# Autodesk Inventor assembly: sweeper
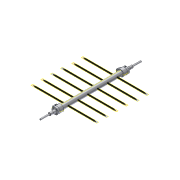
[picture p0: Inventor's stored thumbnail of the model, 180x180]
Saved by Autodesk Inventor 2015 SP1 (Build 190203100, 203)
## iProperties
Created: 2015-01-25
Part Number: sweeper
Document SubType Name: Assembly
Designer: rihoobler
Author: rihoobler
## Documents named in this file (8)
- C:\Users\datenney\Documents\GitHub\CAD\SerenityMk.2\sweeper.iam
- C:\Users\datenney\Documents\GitHub\CAD\SerenityMk.2\Sweeper tube.ipt
- C:\Users\datenney\Documents\GitHub\CAD\SerenityMk.2\Imported Components\tetrix_739077_2012\tetrix_739077_2012.ipt
- C:\Users\datenney\Documents\GitHub\CAD\SerenityMk.2\Imported Components\tetrix_739172_2012\tetrix_739172_2012.iam
- C:\Users\datenney\Documents\GitHub\CAD\SerenityMk.2\Imported Components\tetrix_739088_2012\tetrix_739088_2012.ipt
- C:\Users\datenney\Documents\GitHub\CAD\SerenityMk.2\Imported Components\tetrix_739101_2012\tetrix_739101_2012.ipt
- C:\Users\datenney\Documents\GitHub\CAD\SerenityMk.2\Imported Components\tetrix_739068_2012_288_channel\Part1.ipt
- C:\Users\datenney\Documents\GitHub\CAD\SerenityMk.2\Zip tie start.ipt
## Components (24 placed, 7 different names)
1. Sweeper tube:1 — Insert:1, Insert:2, Mate:40, Mate:47
2. tetrix_739077_2012:1 — Insert:2, Insert:4, Flush:42, Mate:45
3. tetrix_739077_2012:2 — Insert:1, Insert:3, Mate:41, Flush:42, Mate:48, Angle:7, Flush:43
4. tetrix_739172_2012:1 [sub-assembly] — Insert:4, Mate:15, Flush:3, Insert:7, Mate:45
5. tetrix_739172_2012:2 [sub-assembly] — Insert:3, Mate:16, Flush:4, Insert:5, Mate:48
6. tetrix_739088_2012:1 — Mate:16, Flush:4, Angle:7, Angle:8
7. tetrix_739088_2012:2 — Mate:15, Flush:3
8. tetrix_739101_2012:1 — Insert:6
9. tetrix_739101_2012:2 — Insert:5, Insert:6
10. tetrix_739101_2012:3 — Insert:8
11. tetrix_739101_2012:4 — Insert:7, Insert:8
12. Part1:1
13. Zip tie start:1 — Flush:10, Angle:6, Flush:16, Mate:35, Flush:29, Flush:30, Flush:39, Mate:41, Mate:42
14. Zip tie start:2 — Flush:5, Angle:1, Flush:20, Mate:36, Flush:21, Flush:30, Flush:41, Mate:40
15. Zip tie start:3 — Flush:7, Angle:3, Flush:18, Flush:19, Mate:33, Flush:22, Flush:23, Flush:34, Flush:36, Mate:49
16. Zip tie start:4 — Flush:8, Angle:4, Flush:13, Flush:14, Mate:34, Flush:28, Flush:34, Flush:37, Mate:43, Mate:44
17. Zip tie start:5 — Flush:9, Angle:5, Flush:16, Flush:17, Mate:37, Flush:28, Flush:29, Flush:33, Flush:38, Mate:42, Mate:43
18. Zip tie start:6 — Flush:6, Angle:2, Flush:19, Flush:20, Mate:32, Flush:21, Flush:22, Flush:33, Flush:40
19. Zip tie start:7 — Flush:10, Angle:6, Flush:15, Mate:35, Flush:25, Flush:31, Flush:39, Flush:43
20. Zip tie start:8 — Flush:9, Angle:5, Flush:14, Flush:15, Flush:24, Flush:25, Mate:37, Flush:32, Flush:38
21. Zip tie start:9 — Flush:8, Angle:4, Flush:17, Flush:18, Mate:34, Flush:23, Flush:24, Flush:35, Flush:37
22. Zip tie start:10 — Flush:7, Angle:3, Flush:12, Flush:13, Mate:33, Flush:27, Flush:35, Flush:36, Mate:44
23. Zip tie start:11 — Flush:6, Angle:2, Flush:11, Flush:12, Mate:32, Flush:26, Flush:27, Flush:32, Flush:40, Mate:38
24. Zip tie start:12 — Flush:5, Angle:1, Flush:11, Mate:36, Flush:26, Flush:31, Flush:41, Mate:38, Mate:49
## Relationships (75: Flush 41, Mate 18, Insert 8, Angle 8)
- Insert:1: Sweeper tube:1 ↔ tetrix_739077_2012:2
- Insert:2: Sweeper tube:1 ↔ tetrix_739077_2012:1
- Insert:3: tetrix_739077_2012:2 ↔ tetrix_739172_2012:2
- Insert:4: tetrix_739077_2012:1 ↔ tetrix_739172_2012:1
- Mate:15: tetrix_739172_2012:1 ↔ tetrix_739088_2012:2
- Flush:3 (-50.8 mm): tetrix_739172_2012:1 ↔ tetrix_739088_2012:2
- Mate:16: tetrix_739172_2012:2 ↔ tetrix_739088_2012:1
- Flush:4 (-50.8 mm): tetrix_739172_2012:2 ↔ tetrix_739088_2012:1
- Insert:5: tetrix_739172_2012:2 ↔ tetrix_739101_2012:2
- Insert:6: tetrix_739101_2012:1 ↔ tetrix_739101_2012:2
- Insert:7: tetrix_739172_2012:1 ↔ tetrix_739101_2012:4
- Insert:8: tetrix_739101_2012:3 ↔ tetrix_739101_2012:4
- Flush:5: Zip tie start:2 ↔ Zip tie start:12
- Flush:6: Zip tie start:6 ↔ Zip tie start:11
- Flush:7: Zip tie start:3 ↔ Zip tie start:10
- Flush:8: Zip tie start:4 ↔ Zip tie start:9
- Flush:9: Zip tie start:5 ↔ Zip tie start:8
- Flush:10: Zip tie start:1 ↔ Zip tie start:7
- Angle:1 (0 deg): Zip tie start:2 ↔ Zip tie start:12
- Angle:2 (0 deg): Zip tie start:6 ↔ Zip tie start:11
- Angle:3 (0 deg): Zip tie start:3 ↔ Zip tie start:10
- Angle:4 (0 deg): Zip tie start:4 ↔ Zip tie start:9
- Angle:5 (0 deg): Zip tie start:5 ↔ Zip tie start:8
- Angle:6 (0 deg): Zip tie start:1 ↔ Zip tie start:7
- Flush:11: Zip tie start:11 ↔ Zip tie start:12
- Flush:12: Zip tie start:10 ↔ Zip tie start:11
- Flush:13: Zip tie start:4 ↔ Zip tie start:10
- Flush:14: Zip tie start:4 ↔ Zip tie start:8
- Flush:15: Zip tie start:7 ↔ Zip tie start:8
- Flush:16: Zip tie start:1 ↔ Zip tie start:5
- Flush:17: Zip tie start:5 ↔ Zip tie start:9
- Flush:18: Zip tie start:3 ↔ Zip tie start:9
- Flush:19: Zip tie start:3 ↔ Zip tie start:6
- Flush:20: Zip tie start:2 ↔ Zip tie start:6
- Mate:32: Zip tie start:6 ↔ Zip tie start:11
- Mate:33: Zip tie start:3 ↔ Zip tie start:10
- Mate:34: Zip tie start:4 ↔ Zip tie start:9
- Mate:35: Zip tie start:1 ↔ Zip tie start:7
- Mate:36: Zip tie start:2 ↔ Zip tie start:12
- Flush:21 (0.9398 mm): Zip tie start:2 ↔ Zip tie start:6
- Flush:22: Zip tie start:3 ↔ Zip tie start:6
- Flush:23: Zip tie start:3 ↔ Zip tie start:9
- Flush:24: Zip tie start:8 ↔ Zip tie start:9
- Flush:25: Zip tie start:7 ↔ Zip tie start:8
- Mate:37: Zip tie start:5 ↔ Zip tie start:8
- Flush:26: Zip tie start:11 ↔ Zip tie start:12
- Flush:27: Zip tie start:10 ↔ Zip tie start:11
- Flush:28: Zip tie start:4 ↔ Zip tie start:5
- Flush:29: Zip tie start:1 ↔ Zip tie start:5
- Flush:30: Zip tie start:1 ↔ Zip tie start:2
- Flush:31: Zip tie start:7 ↔ Zip tie start:12
- Flush:32: Zip tie start:8 ↔ Zip tie start:11
- Flush:33: Zip tie start:5 ↔ Zip tie start:6
- Flush:34: Zip tie start:3 ↔ Zip tie start:4
- Flush:35: Zip tie start:9 ↔ Zip tie start:10
- Flush:36: Zip tie start:3 ↔ Zip tie start:10
- Flush:37: Zip tie start:4 ↔ Zip tie start:9
- Flush:38: Zip tie start:5 ↔ Zip tie start:8
- Flush:39: Zip tie start:1 ↔ Zip tie start:7
- Flush:40: Zip tie start:6 ↔ Zip tie start:11
- Flush:41: Zip tie start:2 ↔ Zip tie start:12
- Mate:38 (30.3 mm): Zip tie start:11 ↔ Zip tie start:12
- Mate:40: Sweeper tube:1 ↔ Zip tie start:2
- Mate:41 (17.1 mm): tetrix_739077_2012:2 ↔ Zip tie start:1
- Mate:42 (30.2 mm): Zip tie start:1 ↔ Zip tie start:5
- Mate:43 (30.2 mm): Zip tie start:4 ↔ Zip tie start:5
- Mate:44 (30.2 mm): Zip tie start:4 ↔ Zip tie start:10
- Flush:42: tetrix_739077_2012:1 ↔ tetrix_739077_2012:2
- Mate:45: tetrix_739077_2012:1 ↔ tetrix_739172_2012:1
- Mate:47: Sweeper tube:1
- Mate:48: tetrix_739077_2012:2 ↔ tetrix_739172_2012:2
- Angle:7 (0 deg): tetrix_739077_2012:2 ↔ tetrix_739088_2012:1
- Angle:8 (180 deg): tetrix_739088_2012:1
- Flush:43: tetrix_739077_2012:2 ↔ Zip tie start:7
- Mate:49 (30.2 mm): Zip tie start:3 ↔ Zip tie start:12
